# Autodesk Inventor assembly: ExtruderPanel
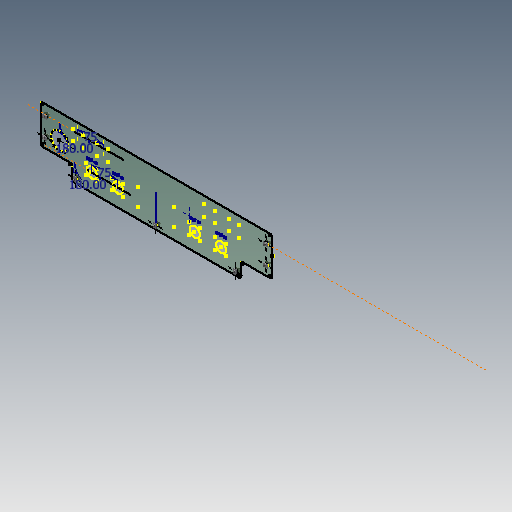
[picture p0: Inventor's stored thumbnail of the model, 512x512]
Saved by Autodesk Inventor 2017 (Build 210142000, 142)
## iProperties
Created: 2016-08-03
Part Number: ExtruderPanel
Document SubType Name: Assembly
Designer: User
Author: User
## Documents named in this file (3)
- C:\Autodesk\SL-Inventor\SL-Beast 3D Printer\ExtruderPanel.iam
- C:\Autodesk\SL-Inventor\SL-Beast 3D Printer\Rear Extruder Panel.ipt
- C:\Autodesk\SL-Inventor\SL-Beast 3D Printer\BoltandTee.iam
## Components (8 placed, 2 different names)
1. Rear Extruder Panel:1
2. BoltandTee:1 [sub-assembly]
3. BoltandTee:2 [sub-assembly]
4. BoltandTee:3 [sub-assembly]
5. BoltandTee:4 [sub-assembly]
6. BoltandTee:5 [sub-assembly]
7. BoltandTee:6 [sub-assembly]
8. BoltandTee:7 [sub-assembly]
## Relationships (7: Insert 7)
- [Insert]: Rear Extruder Panel:1 ↔ BoltandTee:2
- [Insert]: Rear Extruder Panel:1 ↔ BoltandTee:1
- [Insert]: Rear Extruder Panel:1 ↔ BoltandTee:7
- [Insert]: Rear Extruder Panel:1 ↔ BoltandTee:6
- [Insert]: Rear Extruder Panel:1 ↔ BoltandTee:5
- [Insert]: Rear Extruder Panel:1 ↔ BoltandTee:4
- [Insert]: Rear Extruder Panel:1 ↔ BoltandTee:3
